# Autodesk Inventor assembly: Claw
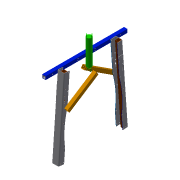
[picture p0: Inventor's stored thumbnail of the model, 180x180]
Saved by Autodesk Inventor 2015 (Build 190159000, 159)
## iProperties
Created: 2015-01-13
Part Number: Claw
Document SubType Name: Assembly
Designer: Collin_2
Author: Collin_2
## Documents named in this file (9)
- T:\FILES\FIRST-Team-1719-CAD-Team\2015 Robot CAD\Devices\Claw\Claw.iam
- T:\FILES\FIRST-Team-1719-CAD-Team\2015 Robot CAD\Devices\Claw\Claw - Base.ipt
- T:\FILES\FIRST-Team-1719-CAD-Team\2015 Robot CAD\Devices\Claw\PC3.5-P1.ipt
- T:\FILES\FIRST-Team-1719-CAD-Team\2015 Robot CAD\Devices\Claw\PC3.5-ROD.ipt
- T:\FILES\FIRST-Team-1719-CAD-Team\2015 Robot CAD\Devices\Claw\Claw - Arm - Top (R).ipt
- T:\FILES\FIRST-Team-1719-CAD-Team\2015 Robot CAD\Devices\Claw\Claw - Arm - Bottom (R).ipt
- T:\FILES\FIRST-Team-1719-CAD-Team\2015 Robot CAD\Devices\Claw\Claw - Arm - Middle.ipt
- T:\FILES\FIRST-Team-1719-CAD-Team\2015 Robot CAD\Devices\Claw\Yarm.ipt
- T:\FILES\FIRST-Team-1719-CAD-Team\2015 Robot CAD\Devices\Claw\Claw - Arm - Plate.ipt
## Components (13 placed, 8 different names)
1. Claw - Base:1 — Mate:18, Mate:19, Mate:20, Mate:21, Tangent:1, Tangent:2, Flush:1
2. PC3.5-P1:1 — Mate:15, Mate:16, Tangent:1, Tangent:2, Flush:1
3. PC3.5-ROD:1 — Mate:15, Mate:16, Angle:1, Mate:37
4. Claw - Arm - Top (R):1 — Mate:20, Mate:21, Mate:26, Mate:27, Angle:1, Mate:38, Mate:43, Insert:4
5. Claw - Arm - Top (R):2 — Mate:23, Mate:24, Mate:31, Mate:35, Mate:45, Flush:5, Insert:3
6. Claw - Arm - Bottom (R):1 — Mate:18, Mate:19, Mate:23, Mate:24, Mate:41, Mate:45, Insert:2, Flush:7
7. Claw - Arm - Bottom (R):2 — Mate:26, Mate:27, Mate:43, Flush:4, Mate:47, Flush:6, Insert:1, Mate:48, Mate:49
8. Claw - Arm - Middle:1 — Mate:31, Mate:41, Flush:5
9. Claw - Arm - Middle:2 — Flush:4, Mate:48, Mate:49
10. Yarm:1 — Mate:35, Mate:37, Mate:40, Insert:3
11. Yarm:2 — Mate:38, Mate:40, Insert:4
12. Claw - Arm - Plate:1 — Mate:47, Flush:6, Insert:1
13. Claw - Arm - Plate:2 — Insert:2, Flush:7
## Relationships (33: Mate 21, Flush 5, Insert 4, Tangent 2, Angle 1)
- Mate:15: PC3.5-P1:1 ↔ PC3.5-ROD:1
- Mate:16: PC3.5-P1:1 ↔ PC3.5-ROD:1
- Mate:18: Claw - Base:1 ↔ Claw - Arm - Bottom (R):1
- Mate:19: Claw - Base:1 ↔ Claw - Arm - Bottom (R):1
- Mate:20: Claw - Base:1 ↔ Claw - Arm - Top (R):1
- Mate:21: Claw - Base:1 ↔ Claw - Arm - Top (R):1
- Mate:23: Claw - Arm - Top (R):2 ↔ Claw - Arm - Bottom (R):1
- Mate:24: Claw - Arm - Top (R):2 ↔ Claw - Arm - Bottom (R):1
- Mate:26: Claw - Arm - Top (R):1 ↔ Claw - Arm - Bottom (R):2
- Mate:27: Claw - Arm - Top (R):1 ↔ Claw - Arm - Bottom (R):2
- Angle:1 (0 deg): PC3.5-ROD:1 ↔ Claw - Arm - Top (R):1
- Mate:31: Claw - Arm - Top (R):2 ↔ Claw - Arm - Middle:1
- Mate:35: Claw - Arm - Top (R):2 ↔ Yarm:1
- Mate:37: PC3.5-ROD:1 ↔ Yarm:1
- Mate:38: Claw - Arm - Top (R):1 ↔ Yarm:2
- Mate:40: Yarm:1 ↔ Yarm:2
- Tangent:1: Claw - Base:1 ↔ PC3.5-P1:1
- Tangent:2 (285.75 mm): Claw - Base:1 ↔ PC3.5-P1:1
- Flush:1 (-114.3 mm): Claw - Base:1 ↔ PC3.5-P1:1
- Mate:41: Claw - Arm - Bottom (R):1 ↔ Claw - Arm - Middle:1
- Mate:43: Claw - Arm - Top (R):1 ↔ Claw - Arm - Bottom (R):2
- Mate:45: Claw - Arm - Top (R):2 ↔ Claw - Arm - Bottom (R):1
- Flush:4: Claw - Arm - Bottom (R):2 ↔ Claw - Arm - Middle:2
- Flush:5: Claw - Arm - Top (R):2 ↔ Claw - Arm - Middle:1
- Mate:47: Claw - Arm - Bottom (R):2 ↔ Claw - Arm - Plate:1
- Flush:6: Claw - Arm - Bottom (R):2 ↔ Claw - Arm - Plate:1
- Insert:1: Claw - Arm - Bottom (R):2 ↔ Claw - Arm - Plate:1
- Insert:2: Claw - Arm - Bottom (R):1 ↔ Claw - Arm - Plate:2
- Flush:7: Claw - Arm - Bottom (R):1 ↔ Claw - Arm - Plate:2
- Mate:48: Claw - Arm - Bottom (R):2 ↔ Claw - Arm - Middle:2
- Mate:49: Claw - Arm - Bottom (R):2 ↔ Claw - Arm - Middle:2
- Insert:3: Claw - Arm - Top (R):2 ↔ Yarm:1
- Insert:4: Claw - Arm - Top (R):1 ↔ Yarm:2
